# Autodesk Inventor assembly: SkeletonDesign
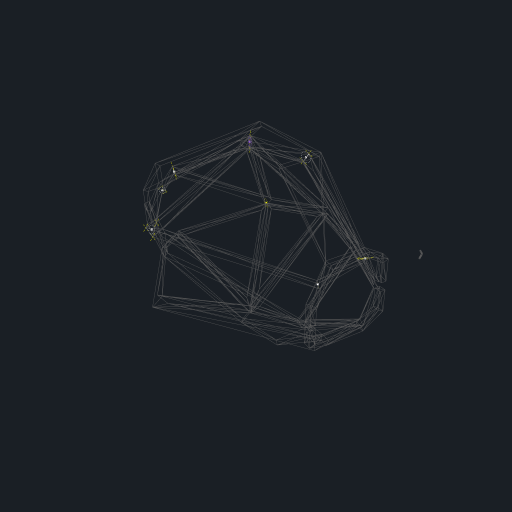
[picture p0: Inventor's stored thumbnail of the model, 512x512]
Saved by Autodesk Inventor 2023 (Build 270158000, 158)
## iProperties
Created: 2023-09-04
Part Number: SkeletonDesign
Document SubType Name: Assembly
Designer: valer
Author: valer
## Documents named in this file (2)
- C:\Users\valer\Desktop\str1ker\cad\Chest\SkeletonDesign.iam
- C:\Users\valer\Desktop\str1ker\cad\Chest\ChestRedesign.ipt
## Components (1 placed, 1 different names)
1. ChestRedesign:1 — Mate:1, Mate:2, Mate:3, Mate:4, Mate:5, Mate:6, Mate:7, Mate:8, Mate:9, Mate:10, Mate:11, Mate:12, Mate:13, Mate:14, Mate:15, Mate:16, Mate:17, Mate:18, Mate:19, Mate:20, Mate:21, Mate:22, Mate:23, Mate:24, Mate:25, Mate:26
## Relationships (27: Mate 26, Flush 1)
- Mate:1: ChestRedesign:1
- Mate:2: ChestRedesign:1
- Mate:3: ChestRedesign:1
- Mate:4: ChestRedesign:1
- Mate:5: ChestRedesign:1
- Mate:6: ChestRedesign:1
- Mate:7: ChestRedesign:1
- Mate:8: ChestRedesign:1
- Mate:9: ChestRedesign:1
- Mate:10: ChestRedesign:1
- Mate:11: ChestRedesign:1
- Mate:12: ChestRedesign:1
- Mate:13: ChestRedesign:1
- Mate:14: ChestRedesign:1
- Flush:1 (-8 mm)
- Mate:15: ChestRedesign:1
- Mate:16: ChestRedesign:1
- Mate:17: ChestRedesign:1
- Mate:18: ChestRedesign:1
- Mate:19: ChestRedesign:1
- Mate:20: ChestRedesign:1
- Mate:21: ChestRedesign:1
- Mate:22: ChestRedesign:1
- Mate:23: ChestRedesign:1
- Mate:24: ChestRedesign:1
- Mate:25: ChestRedesign:1
- Mate:26: ChestRedesign:1
